# Autodesk Inventor assembly: tete_prehension
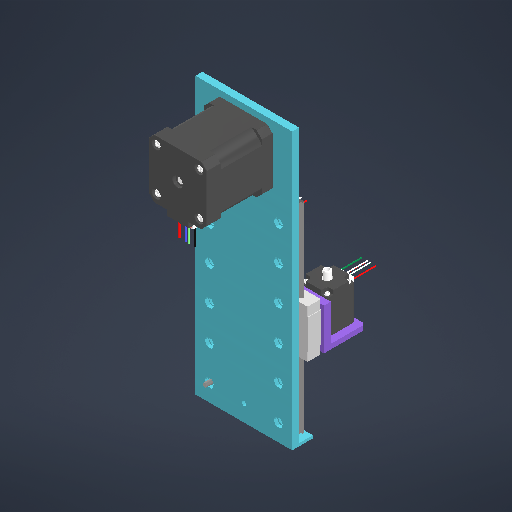
[picture p0: Inventor's stored thumbnail of the model, 512x512]
Saved by Autodesk Inventor 2026 (Build 300175000, 175)
## iProperties
Created: 2025-03-17
Part Number: tete_prehension
Document SubType Name: Assembly
Designer: felix
Author: felix
## Documents named in this file (8)
- C:\Users\malam\Documents\6 - PROJET\14 - PICK&PLACE\Pick-Place\2 - CONCEPTION 3D\20 - CONCEPTION 3D\Tete_Prehension\Workspaces\Espace de travail\tete_prehension.iam
- C:\Users\malam\Documents\6 - PROJET\14 - PICK&PLACE\Pick-Place\2 - CONCEPTION 3D\20 - CONCEPTION 3D\Tete_Prehension\Workspaces\Espace de travail\support_tete_prehension.ipt
- C:\Users\malam\Documents\6 - PROJET\14 - PICK&PLACE\Pick-Place\2 - CONCEPTION 3D\20 - CONCEPTION 3D\Tete_Prehension\Workspaces\Espace de travail\mgn12c_01.ipt
- C:\Users\malam\Documents\6 - PROJET\14 - PICK&PLACE\Pick-Place\2 - CONCEPTION 3D\20 - CONCEPTION 3D\Tete_Prehension\Libraries\Content Center Files\fr-FR\BS EN ISO 4762\BS EN ISO 4762 - M3 x 12(1).ipt
- C:\Users\malam\Documents\6 - PROJET\14 - PICK&PLACE\Pick-Place\2 - CONCEPTION 3D\20 - CONCEPTION 3D\Tete_Prehension\Workspaces\Espace de travail\assemblage_nema8.iam
- C:\Users\malam\Documents\6 - PROJET\14 - PICK&PLACE\Pick-Place\2 - CONCEPTION 3D\20 - CONCEPTION 3D\Tete_Prehension\Workspaces\Espace de travail\assemblage_nema8_gauche.iam
- C:\Users\malam\Documents\6 - PROJET\14 - PICK&PLACE\Pick-Place\2 - CONCEPTION 3D\20 - CONCEPTION 3D\Tete_Prehension\Workspaces\Espace de travail\poulie courroie.ipt
- C:\Users\malam\Documents\6 - PROJET\14 - PICK&PLACE\Pick-Place\2 - CONCEPTION 3D\20 - CONCEPTION 3D\Tete_Prehension\Workspaces\Espace de travail\nema_17.ipt
## Components (10 placed, 7 different names)
1. support_tete_prehension:1 — Mate:2, Mate:3, Mate:4, Mate:5, Mate:6, Mate:7, Mate:10, Mate:11, Mate:12, Mate:13, Mate:14, Mate:15, Mate:21, Mate:22, Mate:23, Mate:24, Mate:25
2. mgn12c_01:1 — Mate:2, Mate:3, Mate:4, Mate:8, Mate:9, Mate:16
3. mgn12c_01:2 — Mate:5, Mate:6, Mate:7, Mate:17
4. BS EN ISO 4762 : Pièce 1 Vis cylindrique à six pans creux - Métrique M3 x 12:1 — Mate:8, Mate:9
5. mgn12c_01:3 — Mate:10, Mate:11, Mate:12, Mate:18, Mate:19
6. mgn12c_01:4 — Mate:13, Mate:14, Mate:15
7. assemblage_nema8:1 [sub-assembly] — Mate:16, Mate:17
8. assemblage_nema8_gauche:1 [sub-assembly] — Mate:18, Mate:19
9. poulie courroie:1 — Mate:21, Mate:22
10. nema_17:1 — Mate:23, Mate:24, Mate:25
## Relationships (23: Mate 23)
- Mate:2: support_tete_prehension:1 ↔ mgn12c_01:1
- Mate:3: support_tete_prehension:1 ↔ mgn12c_01:1
- Mate:4: support_tete_prehension:1 ↔ mgn12c_01:1
- Mate:5: support_tete_prehension:1 ↔ mgn12c_01:2
- Mate:6: support_tete_prehension:1 ↔ mgn12c_01:2
- Mate:7: support_tete_prehension:1 ↔ mgn12c_01:2
- Mate:8: mgn12c_01:1 ↔ BS EN ISO 4762 : Pièce 1 Vis cylindrique à six pans creux - Métrique M3 x 12:1
- Mate:9: mgn12c_01:1 ↔ BS EN ISO 4762 : Pièce 1 Vis cylindrique à six pans creux - Métrique M3 x 12:1
- Mate:10: support_tete_prehension:1 ↔ mgn12c_01:3
- Mate:11: support_tete_prehension:1 ↔ mgn12c_01:3
- Mate:12: support_tete_prehension:1 ↔ mgn12c_01:3
- Mate:13: support_tete_prehension:1 ↔ mgn12c_01:4
- Mate:14: support_tete_prehension:1 ↔ mgn12c_01:4
- Mate:15: support_tete_prehension:1 ↔ mgn12c_01:4
- Mate:16: mgn12c_01:1 ↔ assemblage_nema8:1
- Mate:17: mgn12c_01:2 ↔ assemblage_nema8:1
- Mate:18: mgn12c_01:3 ↔ assemblage_nema8_gauche:1
- Mate:19: mgn12c_01:3 ↔ assemblage_nema8_gauche:1
- Mate:21: support_tete_prehension:1 ↔ poulie courroie:1
- Mate:22: support_tete_prehension:1 ↔ poulie courroie:1
- Mate:23: support_tete_prehension:1 ↔ nema_17:1
- Mate:24: support_tete_prehension:1 ↔ nema_17:1
- Mate:25: support_tete_prehension:1 ↔ nema_17:1
